# Autodesk Inventor assembly: front cortex mount
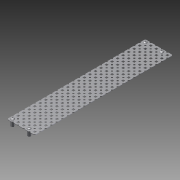
[picture p0: Inventor's stored thumbnail of the model, 180x180]
Saved by Autodesk Inventor 2014 SP1 (Build 180222100, 222)
## iProperties
Created: 2013-09-13
Part Number: front cortex mount
Document SubType Name: Assembly
Designer: Ryan
Author: Ryan
## Documents named in this file (4)
- C:\Users\Ryan\Desktop\sw\toss up 1st A bot\inventor drive\front cortex mount.iam
- C:\Users\Ryan\Desktop\sw\lib\Aperture VEX CAD Library\Metal\Plate\5 x 25.ipt
- C:\Users\Ryan\Desktop\sw\lib\Aperture VEX CAD Library\Standoffs\BEAM-0500.ipt
- C:\Users\Ryan\Desktop\sw\lib\Aperture VEX CAD Library\Hardware\8-32\8-32_.375.ipt
## Components (9 placed, 3 different names)
1. 5 x 25:1 — Mate:1, Mate:3, Mate:4, Mate:5
2. 8-32_.375:1 — Mate:2, Mate:3, Mate:4, Mate:5
3. beam-0500:1 — Mate:1, Mate:2
4. 8-32_.375:2
5. beam-0500:2
6. 8-32_.375:3
7. beam-0500:3
8. 8-32_.375:4
9. beam-0500:4
## Component patterns: (2 elements), (2 elements, first: 8-32_.375:1 + beam-0500:1), Component Pattern 1:2 (2 elements)
## Relationships (5: Mate 5)
- Mate:1: 5 x 25:1 ↔ beam-0500:1
- Mate:2: 8-32_.375:1 ↔ beam-0500:1
- Mate:3: 5 x 25:1 ↔ 8-32_.375:1
- Mate:4 (2.3114 mm): 5 x 25:1 ↔ 8-32_.375:1
- Mate:5 (2.3114 mm): 5 x 25:1 ↔ 8-32_.375:1
## Named parameters: q = 2.3114 mm
